# Autodesk Inventor assembly: Сборка22
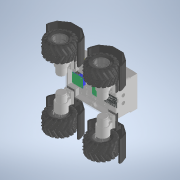
[picture p0: Inventor's stored thumbnail of the model, 180x180]
Saved by Autodesk Inventor 2022 (Build 260153000, 153)
## iProperties
Created: 2023-05-24
Part Number: Сборка22
Document SubType Name: Assembly
Designer: korsh624
Author: korsh624
## Documents named in this file (3)
- C:\git\robot_01\design\Сборка22.iam
- C:\git\robot_01\design\Сборка2.iam
- C:\git\robot_01\design\krish.ipt
## Components (2 placed, 2 different names)
1. Сборка2:1 [sub-assembly] — Заподлицо:1
2. krish:1 — Заподлицо:1
## Relationships (1: Flush 1)
- Заподлицо:1 [Flush]: Сборка2:1 ↔ krish:1
